# Autodesk Inventor assembly: maxon_assembly
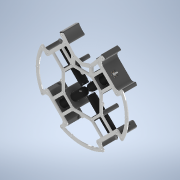
[picture p0: Inventor's stored thumbnail of the model, 180x180]
Saved by Autodesk Inventor 2020 (Build 240168000, 168)
## iProperties
Created: 2024-04-30
Part Number: maxon_assembly
Document SubType Name: Assembly
Designer: 4s
Author: 4s
## Documents named in this file (7)
- C:\Users\4s\Documents\Inventor models\Asterisk\robot_v2\maxon_assembly.iam
- C:\Users\4s\Documents\Inventor models\Asterisk\robot_v2\bottom_plate_v2.ipt
- C:\Users\4s\Documents\Inventor models\Asterisk\robot_v2\maxon mounts\back_mount.ipt
- C:\Users\4s\Documents\Inventor models\Asterisk\robot_v2\maxon mounts\left_mount.ipt
- C:\Users\4s\Documents\Inventor models\Asterisk\robot_v2\maxon mounts\right_mount.ipt
- C:\Users\4s\Documents\Inventor models\Asterisk\robot_v2\maxon motor\maxon motor.iam
- C:\Users\4s\Documents\Inventor models\Asterisk\robot_v2\maxon mounts\inner_mount.ipt
## Components (13 placed, 6 different names)
1. bottom_plate_v2:1 — Совмещение:1, Совмещение:2, Совмещение:3, Совмещение:4, Совмещение:5, Совмещение:6, Совмещение:7, Совмещение:8, Совмещение:9, Совмещение:10, Совмещение:11, Совмещение:12, Совмещение:22, Совмещение:24, Совмещение:26, Совмещение:28
2. back_mount:1 — Совмещение:7, Совмещение:8, Совмещение:9, Совмещение:32, Совмещение:34
3. back_mount:2 — Совмещение:10, Совмещение:11, Совмещение:12, Совмещение:29, Совмещение:33
4. left_mount:1 — Совмещение:4, Совмещение:5, Совмещение:6, Совмещение:31, Совмещение:35
5. right_mount:1 — Совмещение:1, Совмещение:2, Совмещение:3, Совмещение:30, Совмещение:36
6. inner_mount:1 — Совмещение:22, Совмещение:38
7. inner_mount:2 — Совмещение:24, Совмещение:39
8. inner_mount:3 — Совмещение:26, Совмещение:40
9. inner_mount:4 — Совмещение:28, Совмещение:37
10. maxon motor:1 [sub-assembly] — Совмещение:30, Совмещение:36, Совмещение:38
11. maxon motor:2 [sub-assembly] — Совмещение:31, Совмещение:35, Совмещение:39
12. maxon motor:3 [sub-assembly] — Совмещение:32, Совмещение:34, Совмещение:40
13. maxon motor:4 [sub-assembly] — Совмещение:29, Совмещение:33, Совмещение:37
## Relationships (28: Mate 28)
- Совмещение:1 [Mate]: bottom_plate_v2:1 ↔ right_mount:1
- Совмещение:2 [Mate]: bottom_plate_v2:1 ↔ right_mount:1
- Совмещение:3 [Mate]: bottom_plate_v2:1 ↔ right_mount:1
- Совмещение:4 [Mate]: bottom_plate_v2:1 ↔ left_mount:1
- Совмещение:5 [Mate]: bottom_plate_v2:1 ↔ left_mount:1
- Совмещение:6 [Mate]: bottom_plate_v2:1 ↔ left_mount:1
- Совмещение:7 [Mate]: bottom_plate_v2:1 ↔ back_mount:1
- Совмещение:8 [Mate]: bottom_plate_v2:1 ↔ back_mount:1
- Совмещение:9 [Mate]: bottom_plate_v2:1 ↔ back_mount:1
- Совмещение:10 [Mate]: bottom_plate_v2:1 ↔ back_mount:2
- Совмещение:11 [Mate]: bottom_plate_v2:1 ↔ back_mount:2
- Совмещение:12 [Mate]: bottom_plate_v2:1 ↔ back_mount:2
- Совмещение:22 [Mate]: bottom_plate_v2:1 ↔ inner_mount:1
- Совмещение:24 [Mate]: bottom_plate_v2:1 ↔ inner_mount:2
- Совмещение:26 [Mate]: bottom_plate_v2:1 ↔ inner_mount:3
- Совмещение:28 [Mate]: bottom_plate_v2:1 ↔ inner_mount:4
- Совмещение:29 [Mate]: back_mount:2 ↔ maxon motor:4
- Совмещение:30 [Mate]: right_mount:1 ↔ maxon motor:1
- Совмещение:31 [Mate]: left_mount:1 ↔ maxon motor:2
- Совмещение:32 [Mate]: back_mount:1 ↔ maxon motor:3
- Совмещение:33 [Mate]: back_mount:2 ↔ maxon motor:4
- Совмещение:34 [Mate]: back_mount:1 ↔ maxon motor:3
- Совмещение:35 [Mate]: left_mount:1 ↔ maxon motor:2
- Совмещение:36 [Mate]: right_mount:1 ↔ maxon motor:1
- Совмещение:37 [Mate]: inner_mount:4 ↔ maxon motor:4
- Совмещение:38 [Mate]: inner_mount:1 ↔ maxon motor:1
- Совмещение:39 [Mate]: inner_mount:2 ↔ maxon motor:2
- Совмещение:40 [Mate]: inner_mount:3 ↔ maxon motor:3
